# Autodesk Inventor assembly: 42146-03
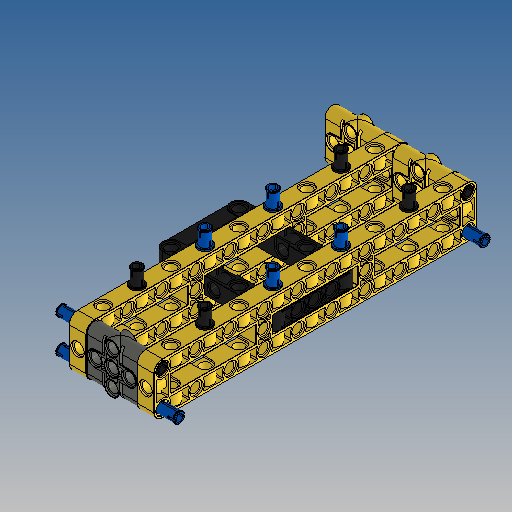
[picture p0: Inventor's stored thumbnail of the model, 512x512]
Saved by Autodesk Inventor 2025 (Build 290162010, 162A)
## iProperties
Created: 2024-11-13
Part Number: 42146-03
Material: Generisch
Document SubType Name: Assembly
Designer: hp.muther
Author: hp.muther
## Documents named in this file (7)
- D:\Inventor\Projekte\Muther\LEGO Technic\LEGO Technik - Raupenkran LR 13000 (42146)\42146-01-03.iam
- D:\Inventor\Projekte\Muther\LEGO Technic\LEGO Pieces\Rahmen, T-Stücke\67491-Yellow.ipt
- D:\Inventor\Projekte\Muther\LEGO Technic\LEGO Pieces\Rahmen, T-Stücke\64179-Black.ipt
- D:\Inventor\Projekte\Muther\LEGO Technic\LEGO Pieces\Pin's\6558-Blue.ipt
- D:\Inventor\Projekte\Muther\LEGO Technic\LEGO Pieces\Pin's\2780-Black.ipt
- D:\Inventor\Projekte\Muther\LEGO Technic\LEGO Pieces\Verbindungselemente\39793-Yellow.ipt
- D:\Inventor\Projekte\Muther\LEGO Technic\LEGO Pieces\Verbindungselemente\39793-LtBluishGray.ipt
## Components (22 placed, 6 different names)
1. 67491-Yellow:1 — Einfügen:1, Passend:1, Einfügen:2, Einfügen:3, Einfügen:12, Passend:2, Einfügen:13, Passend:3, Einfügen:16, Einfügen:19
2. 64179-Black:1 — Einfügen:1, Passend:1
3. 6558-Blue:1 — Einfügen:2
4. 6558-Blue:2 — Einfügen:4, Passend:4, Passend:5
5. 6558-Blue:3 — Einfügen:9, Einfügen:12
6. 6558-Blue:4 — Einfügen:5
7. 6558-Blue:5 — Einfügen:3
8. 2780-Black:1 — Einfügen:7, Passend:2
9. 6558-Blue:6 — Einfügen:17
10. 6558-Blue:7 — Einfügen:10
11. 6558-Blue:8 — Einfügen:11, Einfügen:14
12. 39793-Yellow:1 — Einfügen:21, Passend:5
13. 39793-LtBluishGray:1 — Einfügen:8, Einfügen:9, Einfügen:10, Einfügen:11
14. 67491-Yellow:2 — Einfügen:14, Passend:4, Einfügen:15, Einfügen:17, Einfügen:18, Einfügen:20, Einfügen:21
15. 6558-Blue:9 — Einfügen:18
16. 6558-Blue:10 — Einfügen:6, Einfügen:13
17. 2780-Black:2 — Einfügen:8, Passend:3
18. 2780-Black:3 — Einfügen:16
19. 2780-Black:4 — Einfügen:15
20. 39793-Yellow:2 — Einfügen:4, Einfügen:5, Einfügen:6, Einfügen:7
21. 2780-Black:5 — Einfügen:20
22. 2780-Black:6 — Einfügen:19
## Relationships (26: Insert 21, Mate 5)
- Einfügen:1 [Insert]: 67491-Yellow:1 ↔ 64179-Black:1
- Passend:1 [Mate]: 67491-Yellow:1 ↔ 64179-Black:1
- Einfügen:2 [Insert]: 67491-Yellow:1 ↔ 6558-Blue:1
- Einfügen:3 [Insert]: 67491-Yellow:1 ↔ 6558-Blue:5
- Einfügen:4 [Insert]: 6558-Blue:2 ↔ 39793-Yellow:2
- Einfügen:5 [Insert]: 6558-Blue:4 ↔ 39793-Yellow:2
- Einfügen:6 [Insert]: 6558-Blue:10 ↔ 39793-Yellow:2
- Einfügen:7 [Insert]: 2780-Black:1 ↔ 39793-Yellow:2
- Einfügen:8 [Insert]: 39793-LtBluishGray:1 ↔ 2780-Black:2
- Einfügen:9 [Insert]: 6558-Blue:3 ↔ 39793-LtBluishGray:1
- Einfügen:10 [Insert]: 6558-Blue:7 ↔ 39793-LtBluishGray:1
- Einfügen:11 [Insert]: 6558-Blue:8 ↔ 39793-LtBluishGray:1
- Einfügen:12 [Insert]: 67491-Yellow:1 ↔ 6558-Blue:3
- Passend:2 [Mate]: 67491-Yellow:1 ↔ 2780-Black:1
- Einfügen:13 [Insert]: 67491-Yellow:1 ↔ 6558-Blue:10
- Passend:3 [Mate]: 67491-Yellow:1 ↔ 2780-Black:2
- Einfügen:14 [Insert]: 6558-Blue:8 ↔ 67491-Yellow:2
- Passend:4 [Mate]: 6558-Blue:2 ↔ 67491-Yellow:2
- Einfügen:15 [Insert]: 67491-Yellow:2 ↔ 2780-Black:4
- Einfügen:16 [Insert]: 67491-Yellow:1 ↔ 2780-Black:3
- Einfügen:17 [Insert]: 6558-Blue:6 ↔ 67491-Yellow:2
- Einfügen:18 [Insert]: 67491-Yellow:2 ↔ 6558-Blue:9
- Einfügen:19 [Insert]: 67491-Yellow:1 ↔ 2780-Black:6
- Einfügen:20 [Insert]: 67491-Yellow:2 ↔ 2780-Black:5
- Einfügen:21 [Insert]: 39793-Yellow:1 ↔ 67491-Yellow:2
- Passend:5 [Mate]: 6558-Blue:2 ↔ 39793-Yellow:1
